# Autodesk Inventor assembly: DSA-1x1
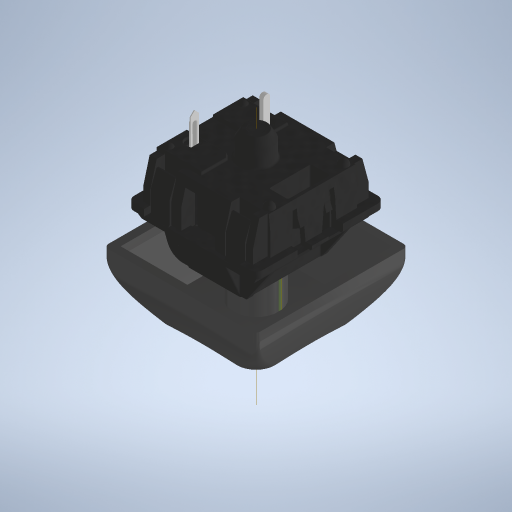
[picture p0: Inventor's stored thumbnail of the model, 512x512]
Saved by Autodesk Inventor 2024.1 (Build 281209000, 209)
## iProperties
Created: 2019-07-03
Part Number: DSA-1x1
Document SubType Name: Assembly
Designer: Thibault
Mass: 0.99122 g
Surface Area: 32.3296 cm^2
Volume: 0.99122 cm^3
Density: 1 g/cm^3
Sending System: Creo  TM  3.0
Author: Thibault
## Documents named in this file (10)
- C:\Users\Thibault\Documents\habilis\mech\mx\DSA-1x1.iam
- C:\Users\Thibault\Documents\habilis\mech\MX_DOWN.ipt
- C:\Users\Thibault\Documents\habilis\mech\MX_UP.ipt
- C:\Users\Thibault\Documents\habilis\mech\MX_PIN.ipt
- C:\Users\Thibault\Documents\habilis\mech\MX_SPRING.ipt
- C:\Users\Thibault\Documents\habilis\mech\MX_CLICK.ipt
- C:\Users\Thibault Polge\Documents\Habilis\mech\mx_stem.ipt
- C:\Users\Thibault\Documents\habilis\mech\keycap_dsa_1x1.ipt
- C:\Users\Thibault\Documents\habilis\mech\mx.iam
- C:\Users\Thibault\Documents\habilis\mech\mx_stem\Brown.ipt
## Components (7 placed, 7 different names)
1. MX_DOWN — Placage:2
2. MX_UP — Placage:3
3. UP_MX — Placage:2, Placage:3, Placage:14, Placage:15, Placage:16
4. MX_PIN
5. MX_SPRING
6. MX_CLICK
7. keycap_dsa_1x1:1 — Placage:14, Placage:15, Placage:16
## Relationships (5: Mate 5)
- Placage:2 [Mate]: MX_DOWN ↔ UP_MX
- Placage:3 [Mate]: MX_UP ↔ UP_MX
- Placage:14 [Mate]: UP_MX ↔ keycap_dsa_1x1:1
- Placage:15 [Mate]: UP_MX ↔ keycap_dsa_1x1:1
- Placage:16 [Mate]: UP_MX ↔ keycap_dsa_1x1:1
